# Autodesk Inventor assembly: Engine skin glued
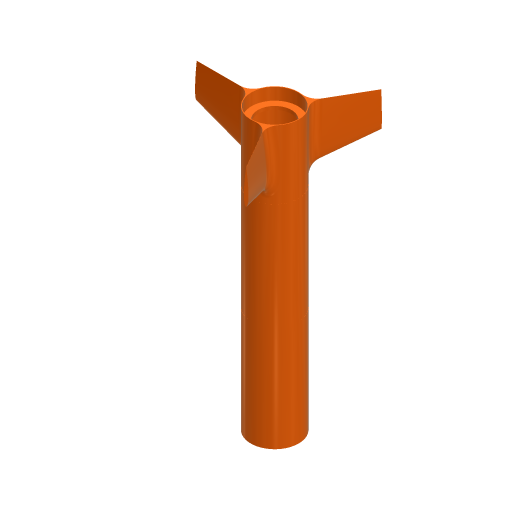
[picture p0: Inventor's stored thumbnail of the model, 512x512]
Saved by Autodesk Inventor 2024 (Build 280153000, 153)
## iProperties
Created: 2024-01-03
Part Number: Engine skin glued
Document SubType Name: Assembly
Designer: Jamie
Mass: 154.6 g
Surface Area: 2298.95 cm^2
Volume: 162.395 cm^3
Density: 0.952 g/cm^3
Author: Jamie
## Documents named in this file (5)
- C:\Users\Jamie\Documents\Uni\DARE\Scrambler-2-CAD\Hide and seek\Engine skin glued.iam
- Engine skin.iam
- C:\Users\Jamie\Documents\Uni\DARE\Scrambler-2-CAD\Hide and seek\Fins.ipt
- C:\Users\Jamie\Documents\Uni\DARE\Scrambler-2-CAD\Hide and seek\Engine lower skin.ipt
- C:\Users\Jamie\Documents\Uni\DARE\Scrambler-2-CAD\Hide and seek\Engine upper skin.ipt
## Components (3 placed, 3 different names)
1. Fins:1 — Mate:1, Mate:2
2. Engine lower skin:1 — Mate:1, Mate:2, Mate:3, Mate:4
3. Engine upper skin:1 — Mate:3, Mate:4
## Relationships (4: Mate 4)
- Mate:1: Fins:1 ↔ Engine lower skin:1
- Mate:2: Fins:1 ↔ Engine lower skin:1
- Mate:3: Engine lower skin:1 ↔ Engine upper skin:1
- Mate:4: Engine lower skin:1 ↔ Engine upper skin:1
